# Autodesk Inventor assembly: robot_1_13
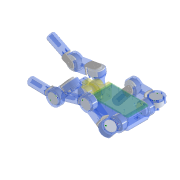
[picture p0: Inventor's stored thumbnail of the model, 180x180]
Saved by Autodesk Inventor 2020 (Build 240168000, 168)
## iProperties
Created: 2021-01-14
Part Number: robot_1_13
Document SubType Name: Assembly
Designer: DELL
Author: DELL
## Documents named in this file (21)
- F:\SoftRobot2.0\FlexipodHardware2.0\FlexipodHardware\Flexipod2.0\robot_2021_2_8\robot.iam
- F:\SoftRobot2.0\FlexipodHardware2.0\FlexipodHardware\Flexipod2.0\RMD_X6_stator.ipt
- F:\SoftRobot2.0\FlexipodHardware2.0\FlexipodHardware\Flexipod2.0\RMD_X6_rotor.ipt
- F:\SoftRobot2.0\FlexipodHardware2.0\FlexipodHardware\Flexipod2.0\Jetson nano v2- Inventor\Jetson_Nano_Dev_Kit_3D_b01.iam
- F:\SoftRobot2.0\FlexipodHardware2.0\FlexipodHardware\Flexipod2.0\battery_6s_1550_ovonic.ipt
- F:\SoftRobot2.0\FlexipodHardware2.0\FlexipodHardware\Flexipod2.0\Arducam Camera.ipt
- F:\SoftRobot2.0\FlexipodHardware2.0\FlexipodHardware\Flexipod2.0\robot_2021_1_28\hip_link_front_mirror.ipt
- F:\SoftRobot2.0\FlexipodHardware2.0\FlexipodHardware\Flexipod2.0\robot_2021_1_28\hip_back_motor_protector.ipt
- F:\SoftRobot2.0\FlexipodHardware2.0\FlexipodHardware\Flexipod2.0\robot_2021_1_28\hard_back_hip_2.ipt
- F:\SoftRobot2.0\FlexipodHardware2.0\FlexipodHardware\Flexipod2.0\robot_2021_1_28\hard_back_hip_2_mirror.ipt
- F:\SoftRobot2.0\FlexipodHardware2.0\FlexipodHardware\Flexipod2.0\robot_2021_2_4\front_hip_mask.ipt
- F:\SoftRobot2.0\FlexipodHardware2.0\FlexipodHardware\Flexipod2.0\robot_2021_2_8\electrical_system_fix_board_2.ipt
- F:\SoftRobot2.0\FlexipodHardware2.0\FlexipodHardware\Flexipod2.0\robot_2021_2_8\battery_fix.ipt
- F:\SoftRobot2.0\FlexipodHardware2.0\FlexipodHardware\Flexipod2.0\robot_2021_2_8\body.ipt
- F:\SoftRobot2.0\FlexipodHardware2.0\FlexipodHardware\Flexipod2.0\robot_2021_2_8\back_hip_cable_protector.ipt
- F:\SoftRobot2.0\FlexipodHardware2.0\FlexipodHardware\Flexipod2.0\robot_2021_2_8\shank_link_2.ipt
- F:\SoftRobot2.0\FlexipodHardware2.0\FlexipodHardware\Flexipod2.0\robot_2021_2_8\shank_thigh_connector.ipt
- F:\SoftRobot2.0\FlexipodHardware2.0\FlexipodHardware\Flexipod2.0\robot_2021_2_8\thigh_hip_connector.ipt
- F:\SoftRobot2.0\FlexipodHardware2.0\FlexipodHardware\Flexipod2.0\robot_2021_2_8\thigh_link.ipt
- F:\SoftRobot2.0\FlexipodHardware2.0\FlexipodHardware\Flexipod2.0\robot_2021_2_8\thigh_link_mirror.ipt
- F:\SoftRobot2.0\FlexipodHardware2.0\FlexipodHardware\Flexipod2.0\robot_2021_2_8\hip_link_front.ipt
## Components (57 placed, 20 different names)
1. body:1 — Flush:30, Flush:31, Flush:32, Mate:372, Mate:373, Mate:375, Mate:376, Mate:378, Mate:379, Mate:380, Mate:381, Mate:382, Mate:383, Mate:388, Mate:389, Angle:16, Mate:396, Mate:397, Angle:18, Mate:399, Mate:400, Angle:19, Angle:20, Angle:21, Angle:28, Angle:29
2. RMD_X6_stator:1 — Mate:1, Flush:4, Mate:251, Mate:364, Mate:365, Mate:366, Mate:375, Mate:376, Mate:396, Mate:397
3. RMD_X6_rotor:1 — Mate:1, Flush:4, Mate:252, Mate:253
4. RMD_X6_stator:2 — Angle:2, Mate:254, Mate:255, Mate:256, Mate:319
5. RMD_X6_rotor:2 — Mate:318, Mate:320
6. RMD_X6_stator:3 — Mate:244, Mate:245, Mate:246
7. RMD_X6_rotor:3 — Mate:348, Mate:350
8. RMD_X6_stator:4 — Mate:284, Mate:378, Mate:379, Mate:380
9. RMD_X6_rotor:4 — Mate:285, Mate:387
10. RMD_X6_stator:6
11. RMD_X6_rotor:6 — Mate:343, Mate:345
12. RMD_X6_rotor:7 — Flush:11, Mate:52, Mate:314, Mate:315
13. RMD_X6_stator:7 — Flush:11, Mate:52, Mate:56, Mate:57, Mate:58, Mate:313
14. RMD_X6_rotor:8 — Mate:51, Flush:10, Mate:53, Mate:54
15. RMD_X6_stator:8 — Mate:51, Flush:10, Mate:55, Mate:361, Mate:363, Mate:372, Mate:373, Mate:399, Mate:400, Mate:401
16. hip_link_front:1 — Mate:53, Mate:54, Mate:55, Mate:56, Mate:57, Mate:58
17. RMD_X6_rotor:9 — Mate:333, Mate:334
18. RMD_X6_stator:9 — Mate:228, Mate:229, Mate:230
19. RMD_X6_rotor:10 — Mate:278
20. RMD_X6_stator:10 — Mate:277, Mate:381, Mate:382, Mate:383
21. Jetson_Nano_Dev_Kit_3D_b01:1 [sub-assembly]
22. battery_6s_1550_ovonic:1 — Mate:360, Angle:15, Flush:29, Mate:390
23. battery_6s_1550_ovonic:2 — Mate:359, Flush:29, Mate:391
24. Arducam Camera:1
25. Arducam Camera:2
26. shank_link_2:9 — Mate:351, Mate:398
27. shank_link_2:10 — Mate:336, Mate:402
28. shank_link_2:11 — Mate:346, Mate:395
29. RMD_X6_rotor:13 — Mate:338, Mate:340
30. RMD_X6_stator:13 — Mate:219, Mate:220, Mate:221
31. shank_link_2:12 — Mate:393, Mate:394
32. RMD_X6_rotor:16 — Mate:328, Mate:330
33. RMD_X6_stator:16 — Mate:274, Mate:275, Mate:279, Mate:329
34. RMD_X6_stator:17 — Mate:266, Mate:267, Mate:268, Mate:324
35. RMD_X6_rotor:17 — Mate:323, Mate:325
36. thigh_link:4 — Mate:219, Mate:220, Mate:221, Mate:331, Mate:332, Mate:339, Angle:16, Angle:25
37. thigh_link:5 — Mate:228, Mate:229, Mate:230, Mate:316, Mate:317, Mate:335, Angle:19, Angle:27, Angle:28
38. thigh_link_mirror:2 — Angle:24
39. thigh_link:6 — Mate:244, Mate:245, Mate:246, Mate:321, Mate:322, Mate:349, Angle:18, Angle:26, Angle:29
40. hip_link_front_mirror:1 — Mate:251, Mate:252, Mate:253, Mate:254, Mate:255, Mate:256
41. hip_back_motor_protector:1 — Mate:266, Mate:267, Mate:268, Mate:286, Mate:287, Mate:288
42. hip_back_motor_protector:2 — Mate:274, Mate:275, Mate:279, Mate:280, Mate:281, Mate:282
43. hard_back_hip_2:1 — Mate:284, Mate:285, Mate:286, Mate:287, Mate:288, Mate:384, Mate:385, Mate:386, Angle:20
44. hard_back_hip_2_mirror:1 — Mate:277, Mate:278, Mate:280, Mate:281, Mate:282, Angle:21
45. thigh_hip_connector:5 — Mate:313, Mate:314, Mate:315, Mate:316, Mate:317
46. thigh_hip_connector:6 — Mate:318, Mate:319, Mate:320, Mate:321, Mate:322
47. thigh_hip_connector:7 — Mate:328, Mate:329, Mate:330, Mate:331, Mate:332
48. thigh_hip_connector:8 — Mate:323, Mate:324, Mate:325
49. shank_thigh_connector:5 — Mate:333, Mate:334, Mate:335, Mate:336, Mate:402, Angle:27
50. shank_thigh_connector:6 — Mate:338, Mate:339, Mate:340, Mate:393, Mate:394, Angle:25
51. shank_thigh_connector:7 — Mate:348, Mate:349, Mate:350, Mate:351, Mate:398, Angle:26
52. shank_thigh_connector:8 — Mate:343, Mate:345, Mate:346, Mate:395, Angle:24
53. electrical_system_fix_board_2:1 — Mate:359, Mate:360, Angle:15, Mate:370, Flush:33, Mate:388, Mate:389, Mate:392
54. front_hip_mask:1 — Mate:361, Mate:363, Mate:401
55. front_hip_mask:2 — Mate:364, Mate:365, Mate:366
56. battery_fix:1 — Mate:370, Mate:390, Mate:391, Mate:392
57. back_hip_cable_protector:1 — Mate:384, Mate:385, Mate:386, Mate:387
## Relationships (155: Mate 124, Flush 17, Angle 14)
- Mate:1: RMD_X6_stator:1 ↔ RMD_X6_rotor:1
- Flush:4 (-3 mm): RMD_X6_stator:1 ↔ RMD_X6_rotor:1
- [Mate]: RMD_X6_stator:2 ↔ RMD_X6_rotor:2
- [Flush] (-3 mm): RMD_X6_stator:2 ↔ RMD_X6_rotor:2
- [Mate]: RMD_X6_stator:3 ↔ RMD_X6_rotor:3
- [Flush] (-3 mm): RMD_X6_stator:3 ↔ RMD_X6_rotor:3
- Angle:2 (180 deg): RMD_X6_stator:2
- [Mate]: RMD_X6_stator:4 ↔ RMD_X6_rotor:4
- [Flush] (-3 mm): RMD_X6_stator:4 ↔ RMD_X6_rotor:4
- [Mate]: RMD_X6_stator:6 ↔ RMD_X6_rotor:6
- [Flush] (-3 mm): RMD_X6_stator:6 ↔ RMD_X6_rotor:6
- Mate:51: RMD_X6_rotor:8 ↔ RMD_X6_stator:8
- Flush:10 (-3 mm): RMD_X6_rotor:8 ↔ RMD_X6_stator:8
- Flush:11 (-3 mm): RMD_X6_rotor:7 ↔ RMD_X6_stator:7
- Mate:52: RMD_X6_rotor:7 ↔ RMD_X6_stator:7
- Mate:53: RMD_X6_rotor:8 ↔ hip_link_front:1
- Mate:54: RMD_X6_rotor:8 ↔ hip_link_front:1
- Mate:55: RMD_X6_stator:8 ↔ hip_link_front:1
- Mate:56: RMD_X6_stator:7 ↔ hip_link_front:1
- Mate:57: RMD_X6_stator:7 ↔ hip_link_front:1
- Mate:58: RMD_X6_stator:7 ↔ hip_link_front:1
- [Mate]: RMD_X6_rotor:9 ↔ RMD_X6_stator:9
- [Flush] (-3 mm): RMD_X6_rotor:9 ↔ RMD_X6_stator:9
- [Mate]: RMD_X6_rotor:10 ↔ RMD_X6_stator:10
- [Flush] (-3 mm): RMD_X6_rotor:10 ↔ RMD_X6_stator:10
- [Mate]: RMD_X6_rotor:13 ↔ RMD_X6_stator:13
- [Flush] (-3 mm): RMD_X6_rotor:13 ↔ RMD_X6_stator:13
- [Flush] (-3 mm): RMD_X6_rotor:16 ↔ RMD_X6_stator:16
- [Mate]: RMD_X6_rotor:16 ↔ RMD_X6_stator:16
- [Mate]: RMD_X6_stator:17 ↔ RMD_X6_rotor:17
- [Flush] (-3 mm): RMD_X6_stator:17 ↔ RMD_X6_rotor:17
- Mate:219: RMD_X6_stator:13 ↔ thigh_link:4
- Mate:220: RMD_X6_stator:13 ↔ thigh_link:4
- Mate:221: RMD_X6_stator:13 ↔ thigh_link:4
- Mate:228: RMD_X6_stator:9 ↔ thigh_link:5
- Mate:229: RMD_X6_stator:9 ↔ thigh_link:5
- Mate:230: RMD_X6_stator:9 ↔ thigh_link:5
- [Mate]: RMD_X6_stator:6 ↔ thigh_link_mirror:2
- [Mate]: RMD_X6_stator:6 ↔ thigh_link_mirror:2
- [Mate]: RMD_X6_stator:6 ↔ thigh_link_mirror:2
- Mate:244: RMD_X6_stator:3 ↔ thigh_link:6
- Mate:245: RMD_X6_stator:3 ↔ thigh_link:6
- Mate:246: RMD_X6_stator:3 ↔ thigh_link:6
- Mate:251: RMD_X6_stator:1 ↔ hip_link_front_mirror:1
- Mate:252: RMD_X6_rotor:1 ↔ hip_link_front_mirror:1
- Mate:253: RMD_X6_rotor:1 ↔ hip_link_front_mirror:1
- Mate:254: RMD_X6_stator:2 ↔ hip_link_front_mirror:1
- Mate:255: RMD_X6_stator:2 ↔ hip_link_front_mirror:1
- Mate:256: RMD_X6_stator:2 ↔ hip_link_front_mirror:1
- Mate:266: RMD_X6_stator:17 ↔ hip_back_motor_protector:1
- Mate:267: RMD_X6_stator:17 ↔ hip_back_motor_protector:1
- Mate:268: RMD_X6_stator:17 ↔ hip_back_motor_protector:1
- Mate:274: RMD_X6_stator:16 ↔ hip_back_motor_protector:2
- Mate:275: RMD_X6_stator:16 ↔ hip_back_motor_protector:2
- Mate:277: RMD_X6_stator:10 ↔ hard_back_hip_2_mirror:1
- Mate:278: RMD_X6_rotor:10 ↔ hard_back_hip_2_mirror:1
- Mate:279: RMD_X6_stator:16 ↔ hip_back_motor_protector:2
- Mate:280: hip_back_motor_protector:2 ↔ hard_back_hip_2_mirror:1
- Mate:281: hip_back_motor_protector:2 ↔ hard_back_hip_2_mirror:1
- Mate:282: hip_back_motor_protector:2 ↔ hard_back_hip_2_mirror:1
- Mate:284: RMD_X6_stator:4 ↔ hard_back_hip_2:1
- Mate:285: RMD_X6_rotor:4 ↔ hard_back_hip_2:1
- Mate:286: hip_back_motor_protector:1 ↔ hard_back_hip_2:1
- Mate:287: hip_back_motor_protector:1 ↔ hard_back_hip_2:1
- Mate:288: hip_back_motor_protector:1 ↔ hard_back_hip_2:1
- Mate:313: RMD_X6_stator:7 ↔ thigh_hip_connector:5
- Mate:314: RMD_X6_rotor:7 ↔ thigh_hip_connector:5
- Mate:315: RMD_X6_rotor:7 ↔ thigh_hip_connector:5
- Mate:316: thigh_link:5 ↔ thigh_hip_connector:5
- Mate:317: thigh_link:5 ↔ thigh_hip_connector:5
- Mate:318: RMD_X6_rotor:2 ↔ thigh_hip_connector:6
- Mate:319: RMD_X6_stator:2 ↔ thigh_hip_connector:6
- Mate:320: RMD_X6_rotor:2 ↔ thigh_hip_connector:6
- Mate:321: thigh_link:6 ↔ thigh_hip_connector:6
- Mate:322: thigh_link:6 ↔ thigh_hip_connector:6
- Mate:323: RMD_X6_rotor:17 ↔ thigh_hip_connector:8
- Mate:324: RMD_X6_stator:17 ↔ thigh_hip_connector:8
- Mate:325: RMD_X6_rotor:17 ↔ thigh_hip_connector:8
- [Mate]: thigh_link_mirror:2 ↔ thigh_hip_connector:8
- [Mate]: thigh_link_mirror:2 ↔ thigh_hip_connector:8
- Mate:328: RMD_X6_rotor:16 ↔ thigh_hip_connector:7
- Mate:329: RMD_X6_stator:16 ↔ thigh_hip_connector:7
- Mate:330: RMD_X6_rotor:16 ↔ thigh_hip_connector:7
- Mate:331: thigh_link:4 ↔ thigh_hip_connector:7
- Mate:332: thigh_link:4 ↔ thigh_hip_connector:7
- Mate:333: RMD_X6_rotor:9 ↔ shank_thigh_connector:5
- Mate:334: RMD_X6_rotor:9 ↔ shank_thigh_connector:5
- Mate:335: thigh_link:5 ↔ shank_thigh_connector:5
- Mate:336: shank_link_2:10 ↔ shank_thigh_connector:5
- Mate:338: RMD_X6_rotor:13 ↔ shank_thigh_connector:6
- Mate:339: thigh_link:4 ↔ shank_thigh_connector:6
- Mate:340: RMD_X6_rotor:13 ↔ shank_thigh_connector:6
- Mate:343: RMD_X6_rotor:6 ↔ shank_thigh_connector:8
- [Mate]: thigh_link_mirror:2 ↔ shank_thigh_connector:8
- Mate:345: RMD_X6_rotor:6 ↔ shank_thigh_connector:8
- Mate:346: shank_link_2:11 ↔ shank_thigh_connector:8
- Mate:348: RMD_X6_rotor:3 ↔ shank_thigh_connector:7
- Mate:349: thigh_link:6 ↔ shank_thigh_connector:7
- Mate:350: RMD_X6_rotor:3 ↔ shank_thigh_connector:7
- Mate:351: shank_link_2:9 ↔ shank_thigh_connector:7
- Mate:359: battery_6s_1550_ovonic:2 ↔ electrical_system_fix_board_2:1
- Mate:360: battery_6s_1550_ovonic:1 ↔ electrical_system_fix_board_2:1
- Angle:15 (0 deg): battery_6s_1550_ovonic:1 ↔ electrical_system_fix_board_2:1
- Flush:29: battery_6s_1550_ovonic:1 ↔ battery_6s_1550_ovonic:2
- Mate:361: RMD_X6_stator:8 ↔ front_hip_mask:1
- Mate:363: RMD_X6_stator:8 ↔ front_hip_mask:1
- Mate:364: RMD_X6_stator:1 ↔ front_hip_mask:2
- Mate:365: RMD_X6_stator:1 ↔ front_hip_mask:2
- Mate:366: RMD_X6_stator:1 ↔ front_hip_mask:2
- Mate:370: electrical_system_fix_board_2:1 ↔ battery_fix:1
- Flush:30: body:1
- Flush:31: body:1
- Flush:32: body:1
- Mate:372: body:1 ↔ RMD_X6_stator:8
- Mate:373: body:1 ↔ RMD_X6_stator:8
- Mate:375: body:1 ↔ RMD_X6_stator:1
- Mate:376: body:1 ↔ RMD_X6_stator:1
- Mate:378: body:1 ↔ RMD_X6_stator:4
- Mate:379: body:1 ↔ RMD_X6_stator:4
- Mate:380: body:1 ↔ RMD_X6_stator:4
- Mate:381: body:1 ↔ RMD_X6_stator:10
- Mate:382: body:1 ↔ RMD_X6_stator:10
- Mate:383: body:1 ↔ RMD_X6_stator:10
- Mate:384: hard_back_hip_2:1 ↔ back_hip_cable_protector:1
- Mate:385: hard_back_hip_2:1 ↔ back_hip_cable_protector:1
- Mate:386: hard_back_hip_2:1 ↔ back_hip_cable_protector:1
- Mate:387: RMD_X6_rotor:4 ↔ back_hip_cable_protector:1
- Flush:33: electrical_system_fix_board_2:1
- Mate:388: body:1 ↔ electrical_system_fix_board_2:1
- Mate:389: body:1 ↔ electrical_system_fix_board_2:1
- Mate:390: battery_6s_1550_ovonic:1 ↔ battery_fix:1
- Mate:391: battery_6s_1550_ovonic:2 ↔ battery_fix:1
- Mate:392: electrical_system_fix_board_2:1 ↔ battery_fix:1
- Angle:16 (0 deg): body:1 ↔ thigh_link:4
- [Angle] (0 deg): body:1 ↔ thigh_link_mirror:2
- Mate:393: shank_link_2:12 ↔ shank_thigh_connector:6
- Mate:394: shank_link_2:12 ↔ shank_thigh_connector:6
- Mate:395: shank_link_2:11 ↔ shank_thigh_connector:8
- Mate:396: body:1 ↔ RMD_X6_stator:1
- Mate:397: body:1 ↔ RMD_X6_stator:1
- Angle:18 (0 deg): body:1 ↔ thigh_link:6
- Mate:398: shank_link_2:9 ↔ shank_thigh_connector:7
- Mate:399: body:1 ↔ RMD_X6_stator:8
- Mate:400: body:1 ↔ RMD_X6_stator:8
- Mate:401: RMD_X6_stator:8 ↔ front_hip_mask:1
- Angle:19 (0 deg): body:1 ↔ thigh_link:5
- Mate:402: shank_link_2:10 ↔ shank_thigh_connector:5
- Angle:20 (320 deg): body:1 ↔ hard_back_hip_2:1
- Angle:21 (80 deg): body:1 ↔ hard_back_hip_2_mirror:1
- Angle:24 (305 deg): thigh_link_mirror:2 ↔ shank_thigh_connector:8
- Angle:25 (320 deg): thigh_link:4 ↔ shank_thigh_connector:6
- Angle:26 (305 deg): thigh_link:6 ↔ shank_thigh_connector:7
- Angle:27 (55 deg): thigh_link:5 ↔ shank_thigh_connector:5
- Angle:28 (270 deg): body:1 ↔ thigh_link:5
- Angle:29 (305 deg): body:1 ↔ thigh_link:6
## Named parameters: d11_d3 = 0 mm, d12_d4 = -3 mm, d13_d3 = 0 mm, d14_d4 = -3 mm, d32_d13_d3 = 0 mm, d33_d14_d4 = -3 mm, d36_d13_d3 = 0 mm, d37_d14_d4 = -3 mm, d79_d64 = 0 mm, d80_d65 = -3 mm, d81_d64 = 0 mm, d82_d65 = -3 mm, d244_d79_d64 = 0 mm, d245_d80_d65 = -3 mm, d258_d66 = -3 mm, d259_d67 = 0 mm, d260_d11_d3 = 0 mm, d261_d12_d4 = -3 mm
